# Autodesk Inventor assembly: DoorAssembly
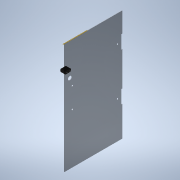
[picture p0: Inventor's stored thumbnail of the model, 180x180]
Saved by Autodesk Inventor 2021.3 (Build 253353000, 353)
## iProperties
Created: 2021-05-13
Part Number: DoorAssembly
Document SubType Name: Assembly
Designer: gisen
Author: gisen
## Documents named in this file (3)
- C:\Users\gisen\GitProjects\CAD-Data\CuboidAccessories\SecurityBox\Assemblies\DoorAssembly.iam
- C:\Users\gisen\GitProjects\CAD-Data\CuboidAccessories\SecurityBox\3DPrintedParts\DoorLockHook.ipt
- C:\Users\gisen\GitProjects\CAD-Data\CuboidAccessories\SecurityBox\Plates\DoorPlateLower.ipt
## Components (2 placed, 2 different names)
1. DoorLockHook:1 — メイト:10, メイト:11, メイト:12
2. DoorPlateLower:1 — メイト:7, メイト:8, メイト:9, メイト:10, メイト:11, メイト:12
## Relationships (6: Mate 6)
- メイト:7 [Mate]: DoorPlateLower:1
- メイト:8 [Mate]: DoorPlateLower:1
- メイト:9 [Mate]: DoorPlateLower:1
- メイト:10 [Mate]: DoorLockHook:1 ↔ DoorPlateLower:1
- メイト:11 [Mate]: DoorLockHook:1 ↔ DoorPlateLower:1
- メイト:12 [Mate]: DoorLockHook:1 ↔ DoorPlateLower:1
